# Autodesk Inventor assembly: Assembly2
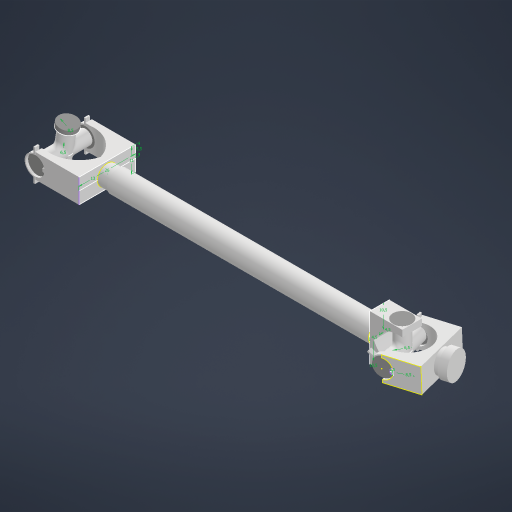
[picture p0: Inventor's stored thumbnail of the model, 512x512]
Saved by Autodesk Inventor 2023 (Build 270158030, 158C)
## iProperties
Created: 2023-02-03
Part Number: Assembly2
Document SubType Name: Assembly
Designer: Monster
Author: Monster
## Documents named in this file (6)
- C:\Users\Monster\Desktop\Ders\UKA\shaft toplam\shaft imalat vida\Assembly2 vidalı.iam
- C:\Users\Monster\Desktop\Ders\UKA\shaft toplam\shaft imalat vida\Part1.ipt
- C:\Users\Monster\Desktop\Ders\UKA\shaft toplam\shaft imalat vida\Part5.ipt
- C:\Users\Monster\Desktop\Ders\UKA\shaft toplam\shaft imalat vida\Part3.ipt
- C:\Users\Monster\Desktop\Ders\UKA\shaft toplam\shaft imalat vida\shaft 4 kol.ipt
- C:\Users\Monster\Desktop\Ders\UKA\shaft toplam\shaft imalat vida\vida.ipt
## Components (16 placed, 5 different names)
1. Part1:1 — Mate:9, Mate:11, Mate:21, Mate:26, Mate:35, Flush:1
2. Part5:1 — Mate:36, Mate:37, Mate:38, Flush:2, Mate:39, Flush:3
3. Part3:1 — Mate:9
4. Part3:2 — Mate:11
5. shaft 4 kol:1 — Mate:27, Mate:28, Mate:29, Mate:30, Mate:31, Mate:32, Mate:33, Mate:34, Mate:35, Mate:36
6. shaft 4 kol:2 — Mate:17, Mate:18, Mate:19, Mate:20, Mate:22, Mate:23, Mate:24, Mate:25
7. vida:1 — Mate:17, Mate:18
8. vida:2 — Mate:24, Mate:25
9. vida:3 — Mate:22, Mate:23, Mate:26
10. vida:4 — Mate:19, Mate:20, Mate:21
11. vida:5 — Mate:27, Mate:28, Flush:1
12. vida:6 — Mate:31, Mate:32
13. vida:7 — Mate:29, Mate:33
14. vida:8 — Mate:30, Mate:34, Mate:37
15. Part3:3 — Mate:38, Flush:2
16. Part3:4 — Mate:39, Flush:3
## Relationships (28: Mate 25, Flush 3)
- Mate:9: Part1:1 ↔ Part3:1
- Mate:11: Part1:1 ↔ Part3:2
- Mate:17: shaft 4 kol:2 ↔ vida:1
- Mate:18: shaft 4 kol:2 ↔ vida:1
- Mate:19: shaft 4 kol:2 ↔ vida:4
- Mate:20: shaft 4 kol:2 ↔ vida:4
- Mate:21: Part1:1 ↔ vida:4
- Mate:22: shaft 4 kol:2 ↔ vida:3
- Mate:23: shaft 4 kol:2 ↔ vida:3
- Mate:24: shaft 4 kol:2 ↔ vida:2
- Mate:25: shaft 4 kol:2 ↔ vida:2
- Mate:26: Part1:1 ↔ vida:3
- Mate:27: shaft 4 kol:1 ↔ vida:5
- Mate:28: shaft 4 kol:1 ↔ vida:5
- Mate:29: shaft 4 kol:1 ↔ vida:7
- Mate:30: shaft 4 kol:1 ↔ vida:8
- Mate:31: shaft 4 kol:1 ↔ vida:6
- Mate:32: shaft 4 kol:1 ↔ vida:6
- Mate:33: shaft 4 kol:1 ↔ vida:7
- Mate:34: shaft 4 kol:1 ↔ vida:8
- Mate:35: Part1:1 ↔ shaft 4 kol:1
- Flush:1: Part1:1 ↔ vida:5
- Mate:36: Part5:1 ↔ shaft 4 kol:1
- Mate:37: Part5:1 ↔ vida:8
- Mate:38: Part5:1 ↔ Part3:3
- Flush:2 (-1 mm): Part5:1 ↔ Part3:3
- Mate:39: Part5:1 ↔ Part3:4
- Flush:3 (-1 mm): Part5:1 ↔ Part3:4
